# Autodesk Inventor assembly: Weight Assembly
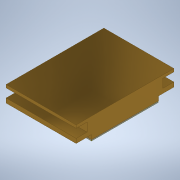
[picture p0: Inventor's stored thumbnail of the model, 180x180]
Saved by Autodesk Inventor 2022 (Build 260153000, 153)
## iProperties
Created: 2021-03-04
Part Number: Weight Assembly
Document SubType Name: Assembly
Designer: caleb
Author: caleb
## Documents named in this file (3)
- C:\Users\Caleb\Desktop\nebraska-silicon-lab\Hardware\ETL\Module Assembly\Weight - V2\Weight Assembly - V2.iam
- C:\Users\Caleb\Desktop\nebraska-silicon-lab\Hardware\ETL\Module Assembly\Weight - V2\Weight Body - V2.ipt
- C:\Users\Caleb\Desktop\nebraska-silicon-lab\Hardware\ETL\Module Assembly\Weight - V2\Bottom Surface - V2.ipt
## Components (2 placed, 2 different names)
1. Weight Body - V2:1 — Insert:1
2. Bottom Surface - V2:1 — Insert:1
## Relationships (1: Insert 1)
- Insert:1: Weight Body - V2:1 ↔ Bottom Surface - V2:1
